# Autodesk Inventor assembly: POM_T5_34
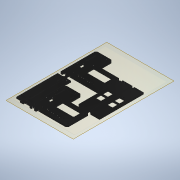
[picture p0: Inventor's stored thumbnail of the model, 180x180]
Saved by Autodesk Inventor 2020 (Build 240168000, 168)
## iProperties
Created: 2021-08-27
Part Number: POM_T5_34
Document SubType Name: Assembly
Designer: Masato
Author: Masato
## Documents named in this file (5)
- C:\Inventor\SUSTAINA-OP\Cam\POM_T5_34.iam
- C:\Inventor\SUSTAINA-OP\Cam\DisposableBoard.ipt
- C:\Inventor\SUSTAINA-OP\UpperBody\Cockpit\Cockpit_top_frame.ipt
- C:\Inventor\SUSTAINA-OP\UpperBody\Cockpit\Cockpit_side_frame.ipt
- C:\Inventor\SUSTAINA-OP\UpperBody\Cockpit\Cockpit_battery_bottom_frame.ipt
## Components (6 placed, 4 different names)
1. DisposableBoard:1 — メイト:2, メイト:1, フラッシュ:1, フラッシュ:2, メイト:22, メイト:36, メイト:37, メイト:38, フラッシュ:3, フラッシュ:4
2. Cockpit_side_frame:1 — メイト:36, フラッシュ:6, メイト:40, メイト:42
3. Cockpit_battery_bottom_frame:1 — メイト:37, フラッシュ:3, フラッシュ:4, フラッシュ:5, メイト:39, フラッシュ:6, メイト:40
4. Cockpit_side_frame:2 — メイト:38, フラッシュ:5, メイト:39, メイト:43
5. Cockpit_top_frame:1 — メイト:22, メイト:42, メイト:43
6. Cockpit_top_frame:3
## Component patterns: (2 elements, first: Cockpit_top_frame:1)
## Relationships (16: Mate 10, Flush 6)
- メイト:2 [Mate]: DisposableBoard:1
- メイト:1 [Mate]: DisposableBoard:1
- フラッシュ:1 [Flush]: DisposableBoard:1
- フラッシュ:2 [Flush]: DisposableBoard:1
- メイト:22 [Mate]: DisposableBoard:1 ↔ Cockpit_top_frame:1
- メイト:36 [Mate]: DisposableBoard:1 ↔ Cockpit_side_frame:1
- メイト:37 [Mate]: DisposableBoard:1 ↔ Cockpit_battery_bottom_frame:1
- メイト:38 [Mate]: DisposableBoard:1 ↔ Cockpit_side_frame:2
- フラッシュ:3 [Flush] (2 mm): DisposableBoard:1 ↔ Cockpit_battery_bottom_frame:1
- フラッシュ:4 [Flush] (2 mm): DisposableBoard:1 ↔ Cockpit_battery_bottom_frame:1
- フラッシュ:5 [Flush]: Cockpit_battery_bottom_frame:1 ↔ Cockpit_side_frame:2
- メイト:39 [Mate] (2.5 mm): Cockpit_battery_bottom_frame:1 ↔ Cockpit_side_frame:2
- フラッシュ:6 [Flush]: Cockpit_side_frame:1 ↔ Cockpit_battery_bottom_frame:1
- メイト:40 [Mate] (2.5 mm): Cockpit_side_frame:1 ↔ Cockpit_battery_bottom_frame:1
- メイト:42 [Mate] (2.5 mm): Cockpit_side_frame:1 ↔ Cockpit_top_frame:1
- メイト:43 [Mate] (2.5 mm): Cockpit_side_frame:2 ↔ Cockpit_top_frame:1
